# Autodesk Inventor assembly: SMALLER
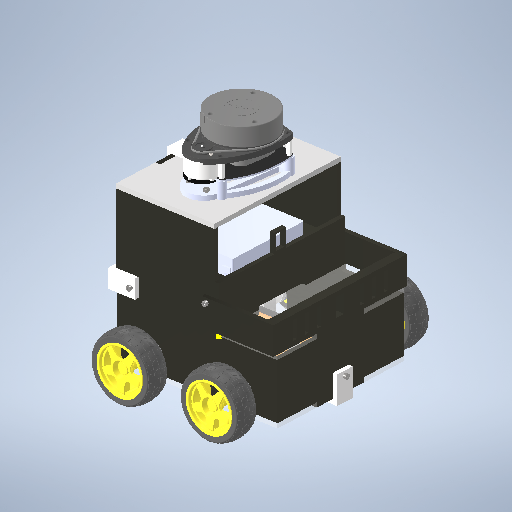
[picture p0: Inventor's stored thumbnail of the model, 512x512]
Saved by Autodesk Inventor 2025.3 (Build 293356030, 356C)
## iProperties
Created: 2026-06-30
Part Number: SMALLER
Document SubType Name: Assembly
Designer: user
Author: user
## Documents named in this file (14)
- C:\Docs\shcool\dojo\Design_3\Smaller\SMALLER.iam
- C:\Docs\shcool\dojo\Design_3\Smaller\WHEEL_BASE.iam
- C:\Docs\shcool\dojo\Design_3\Smaller\back.ipt
- C:\Docs\shcool\dojo\Design_3\Smaller\Fastener.ipt
- C:\Docs\shcool\dojo\Design_3\Smaller\SIDE_1.ipt
- C:\Docs\shcool\dojo\Design_3\Smaller\HOOD_1.ipt
- C:\Docs\shcool\dojo\Design_3\Smaller\TOP_1.ipt
- C:\Docs\shcool\dojo\Design_3\Smaller\FRONT_1.ipt
- C:\Docs\shcool\dojo\Design_3\Smaller\COVER_1.ipt
- C:\Docs\shcool\dojo\Design_3\Smaller\BONNET.ipt
- C:\Docs\shcool\dojo\Design_3\lidar_assembly\assembled_lidar.iam
- C:\Docs\shcool\dojo\Design_3\pi_internals\Complete_model.iam
- C:\Users\user\OneDrive\Documents\Inventor\Content Center Files\R2025\en-US\ISO 4762(2)\ISO 4762 - M3 x 16ISO.ipt
- C:\Users\user\OneDrive\Documents\Inventor\Content Center Files\R2025\en-US\ISO 7040\DIEN EN ISO 7040 - M3.ipt
## Components (43 placed, 13 different names)
1. WHEEL_BASE:1 [sub-assembly] — Mate:15, Mate:16, Mate:17, Mate:18, Mate:19
2. back:1 — Mate:5, Mate:6, Mate:7, Mate:8, Mate:9, Mate:12, Mate:14, Mate:15, Mate:21, Mate:23, Mate:24, Mate:25, Mate:26, Mate:27, Mate:28, Insert:23, Insert:24, Insert:25
3. SIDE_1:1 — Mate:5, Mate:6, Mate:7, Mate:13, Mate:32, Mate:33, Insert:6
4. SIDE_1:2 — Mate:8, Mate:9, Mate:16, Mate:20, Mate:22, Mate:38, Insert:4
5. Fastener:2 — Mate:20, Mate:21, Mate:22, Insert:10, Insert:13
6. Fastener:3 — Mate:12, Mate:13, Mate:14, Insert:7, Insert:8, Insert:11
7. Fastener:4 — Mate:17, Mate:18, Mate:19, Insert:14, Insert:27
8. HOOD_1:1 — Mate:23, Mate:24, Mate:30, Mate:31, Mate:37
9. TOP_1:1 — Mate:25, Mate:26, Mate:29, Mate:44, Mate:45, Insert:19, Insert:20, Insert:21, Insert:22
10. Fastener:5 — Mate:27, Mate:28, Mate:29, Insert:9, Insert:12
11. FRONT_1:1 — Mate:30, Mate:31, Mate:34, Mate:35, Mate:36, Flush:1, Insert:2
12. COVER_1:1 — Mate:32, Mate:33, Mate:42, Mate:43
13. Fastener:6 — Mate:34, Mate:35, Mate:36, Insert:1, Insert:26
14. BONNET:1 — Mate:37, Flush:1, Mate:38, Insert:3, Insert:5
15. Complete_model:1 [sub-assembly] — Mate:42, Mate:43
16. ISO 4762 M3 x 16:1 — Insert:1
17. DIN EN ISO 7040 M3:1 — Insert:2
18. ISO 4762 M3 x 16:2 — Insert:5
19. DIN EN ISO 7040 M3:2 — Insert:4
20. ISO 4762 M3 x 16:3 — Insert:3
21. DIN EN ISO 7040 M3:3 — Insert:8
22. ISO 4762 M3 x 16:4 — Insert:11
23. DIN EN ISO 7040 M3:4 — Insert:19
24. ISO 4762 M3 x 16:5 — Insert:7
25. DIN EN ISO 7040 M3:5 — Insert:23
26. ISO 4762 M3 x 16:6 — Insert:10
27. DIN EN ISO 7040 M3:6 — Insert:6
28. ISO 4762 M3 x 16:7 — Insert:9
29. ISO 4762 M3 x 16:8 — Insert:12
30. ISO 4762 M3 x 16:9 — Insert:13
31. ISO 4762 M3 x 16:10 — Insert:14
32. ISO 4762 M3 x 16:11 — Insert:15
33. ISO 4762 M3 x 16:12 — Insert:16
34. ISO 4762 M3 x 16:15 — Insert:17
35. ISO 4762 M3 x 16:16 — Insert:26
36. ISO 4762 M3 x 16:21 — Insert:27
37. ISO 4762 M3 x 16:22 — Insert:18
38. assembled_lidar:1 [sub-assembly] — Mate:44, Mate:45, Insert:15, Insert:16, Insert:17, Insert:18
39. DIN EN ISO 7040 M3:7 — Insert:24
40. DIN EN ISO 7040 M3:8 — Insert:22
41. DIN EN ISO 7040 M3:9 — Insert:21
42. DIN EN ISO 7040 M3:10 — Insert:20
43. DIN EN ISO 7040 M3:24 — Insert:25
## Relationships (64: Mate 36, Insert 27, Flush 1)
- Mate:5: back:1 ↔ SIDE_1:1
- Mate:6: back:1 ↔ SIDE_1:1
- Mate:7: back:1 ↔ SIDE_1:1
- Mate:8: back:1 ↔ SIDE_1:2
- Mate:9: back:1 ↔ SIDE_1:2
- Mate:12: back:1 ↔ Fastener:3
- Mate:13: SIDE_1:1 ↔ Fastener:3
- Mate:14: back:1 ↔ Fastener:3
- Mate:15: WHEEL_BASE:1 ↔ back:1
- Mate:16: WHEEL_BASE:1 ↔ SIDE_1:2
- Mate:17: WHEEL_BASE:1 ↔ Fastener:4
- Mate:18: WHEEL_BASE:1 ↔ Fastener:4
- Mate:19: WHEEL_BASE:1 ↔ Fastener:4
- Mate:20: SIDE_1:2 ↔ Fastener:2
- Mate:21: back:1 ↔ Fastener:2
- Mate:22: SIDE_1:2 ↔ Fastener:2
- Mate:23: back:1 ↔ HOOD_1:1
- Mate:24: back:1 ↔ HOOD_1:1
- Mate:25: back:1 ↔ TOP_1:1
- Mate:26: back:1 ↔ TOP_1:1
- Mate:27: back:1 ↔ Fastener:5
- Mate:28: back:1 ↔ Fastener:5
- Mate:29: TOP_1:1 ↔ Fastener:5
- Mate:30: HOOD_1:1 ↔ FRONT_1:1
- Mate:31: HOOD_1:1 ↔ FRONT_1:1
- Mate:32: SIDE_1:1 ↔ COVER_1:1
- Mate:33: SIDE_1:1 ↔ COVER_1:1
- Mate:34: FRONT_1:1 ↔ Fastener:6
- Mate:35: FRONT_1:1 ↔ Fastener:6
- Mate:36: FRONT_1:1 ↔ Fastener:6
- Mate:37: HOOD_1:1 ↔ BONNET:1
- Flush:1: FRONT_1:1 ↔ BONNET:1
- Mate:38: SIDE_1:2 ↔ BONNET:1
- Mate:42: COVER_1:1 ↔ Complete_model:1
- Mate:43: COVER_1:1 ↔ Complete_model:1
- Insert:1: Fastener:6 ↔ ISO 4762 M3 x 16:1
- Insert:2: FRONT_1:1 ↔ DIN EN ISO 7040 M3:1
- Insert:3: BONNET:1 ↔ ISO 4762 M3 x 16:3
- Insert:4: SIDE_1:2 ↔ DIN EN ISO 7040 M3:2
- Insert:5: BONNET:1 ↔ ISO 4762 M3 x 16:2
- Insert:6: SIDE_1:1 ↔ DIN EN ISO 7040 M3:6
- Insert:7: Fastener:3 ↔ ISO 4762 M3 x 16:5
- Insert:8: Fastener:3 ↔ DIN EN ISO 7040 M3:3
- Insert:9: Fastener:5 ↔ ISO 4762 M3 x 16:7
- Insert:10: Fastener:2 ↔ ISO 4762 M3 x 16:6
- Insert:11: Fastener:3 ↔ ISO 4762 M3 x 16:4
- Insert:12: Fastener:5 ↔ ISO 4762 M3 x 16:8
- Insert:13: Fastener:2 ↔ ISO 4762 M3 x 16:9
- Insert:14: Fastener:4 ↔ ISO 4762 M3 x 16:10
- Mate:44: TOP_1:1 ↔ assembled_lidar:1
- Mate:45: TOP_1:1 ↔ assembled_lidar:1
- Insert:15: ISO 4762 M3 x 16:11 ↔ assembled_lidar:1
- Insert:16: ISO 4762 M3 x 16:12 ↔ assembled_lidar:1
- Insert:17: ISO 4762 M3 x 16:15 ↔ assembled_lidar:1
- Insert:18: ISO 4762 M3 x 16:22 ↔ assembled_lidar:1
- Insert:19: TOP_1:1 ↔ DIN EN ISO 7040 M3:4
- Insert:20: TOP_1:1 ↔ DIN EN ISO 7040 M3:10
- Insert:21: TOP_1:1 ↔ DIN EN ISO 7040 M3:9
- Insert:22: TOP_1:1 ↔ DIN EN ISO 7040 M3:8
- Insert:23: back:1 ↔ DIN EN ISO 7040 M3:5
- Insert:24: back:1 ↔ DIN EN ISO 7040 M3:7
- Insert:25: back:1 ↔ DIN EN ISO 7040 M3:24
- Insert:26: Fastener:6 ↔ ISO 4762 M3 x 16:16
- Insert:27: Fastener:4 ↔ ISO 4762 M3 x 16:21
